# Autodesk Inventor assembly: Конвейр сборка
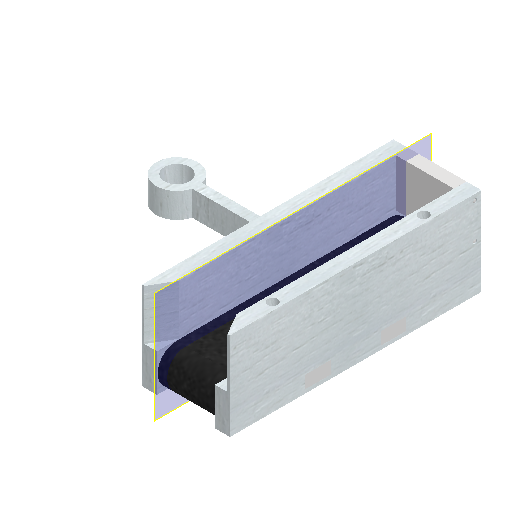
[picture p0: Inventor's stored thumbnail of the model, 512x512]
Saved by Autodesk Inventor 2022 (Build 260153000, 153)
## iProperties
Created: 2023-02-19
Part Number: Конвейр сборка
Document SubType Name: Assembly
Designer: Глеб
Mass: 469.366 g
Surface Area: 1644.22 cm^2
Volume: 465.137 cm^3
Density: 1.00909 g/cm^3
Author: Глеб
## Documents named in this file (9)
- C:\Users\Глеб\Documents\Inventor\Файлы Inventor\Конвейр сборка.iam
- C:\Users\Глеб\Documents\Inventor\Файлы Inventor\Конвейр без шпилек сборка.iam
- C:\Users\Глеб\Documents\Inventor\Файлы Inventor\Шпилька скрепления деталей.ipt
- C:\Users\Глеб\Documents\Inventor\Файлы Inventor\GearMotor\Motor.iam
- C:\Users\Глеб\Documents\Inventor\Файлы Inventor\Шкив для ДПТ.ipt
- C:\Users\Глеб\Documents\Inventor\Файлы Inventor\MX1508.ipt
- C:\Users\Глеб\Documents\Inventor\Файлы Inventor\Стенка конвейера задняя.ipt
- C:\Users\Глеб\Documents\Inventor\Файлы Inventor\Ременная передача.ipt
- C:\Users\Глеб\Documents\Inventor\Файлы Inventor\Лента конвейера.ipt
## Components (9 placed, 8 different names)
1. Лента конвейера:1 — Совмещение:25, Совмещение:26
2. Конвейр без шпилек сборка:1 [sub-assembly] — Совмещение:1, Совмещение:4, Совмещение:7, Совмещение:12, Заподлицо:8, Заподлицо:9, Заподлицо:18, Заподлицо:19, Совмещение:16, Совмещение:19, Совмещение:21, Совмещение:23, Совмещение:24, Совмещение:25
3. Шпилька скрепления деталей:1 — Совмещение:1, Заподлицо:19
4. Шпилька скрепления деталей:3 — Совмещение:4, Заподлицо:18
5. GearMotor:1 [sub-assembly] — Совмещение:16, Совмещение:18, Совмещение:19
6. Шкив для ДПТ:1 — Совмещение:15, Заподлицо:17, Совмещение:18
7. MX1508:1 — Совмещение:7, Совмещение:23, Совмещение:24
8. Стенка конвейера задняя:1 — Совмещение:12, Заподлицо:8, Заподлицо:9, Совмещение:26
9. Ременная передача:1 — Совмещение:15, Заподлицо:17, Совмещение:21
## Relationships (18: Mate 13, Flush 5)
- Совмещение:1 [Mate]: Конвейр без шпилек сборка:1 ↔ Шпилька скрепления деталей:1
- Совмещение:4 [Mate]: Конвейр без шпилек сборка:1 ↔ Шпилька скрепления деталей:3
- Совмещение:7 [Mate] (1 mm): Конвейр без шпилек сборка:1 ↔ MX1508:1
- Совмещение:12 [Mate]: Конвейр без шпилек сборка:1 ↔ Стенка конвейера задняя:1
- Заподлицо:8 [Flush]: Конвейр без шпилек сборка:1 ↔ Стенка конвейера задняя:1
- Заподлицо:9 [Flush]: Конвейр без шпилек сборка:1 ↔ Стенка конвейера задняя:1
- Совмещение:15 [Mate]: Шкив для ДПТ:1 ↔ Ременная передача:1
- Заподлицо:17 [Flush]: Шкив для ДПТ:1 ↔ Ременная передача:1
- Заподлицо:18 [Flush]: Конвейр без шпилек сборка:1 ↔ Шпилька скрепления деталей:3
- Заподлицо:19 [Flush]: Конвейр без шпилек сборка:1 ↔ Шпилька скрепления деталей:1
- Совмещение:16 [Mate] (3 mm): Конвейр без шпилек сборка:1 ↔ GearMotor:1
- Совмещение:18 [Mate]: GearMotor:1 ↔ Шкив для ДПТ:1
- Совмещение:19 [Mate] (2 mm): Конвейр без шпилек сборка:1 ↔ GearMotor:1
- Совмещение:21 [Mate]: Конвейр без шпилек сборка:1 ↔ Ременная передача:1
- Совмещение:23 [Mate] (2 mm): Конвейр без шпилек сборка:1 ↔ MX1508:1
- Совмещение:24 [Mate]: Конвейр без шпилек сборка:1 ↔ MX1508:1
- Совмещение:25 [Mate]: Лента конвейера:1 ↔ Конвейр без шпилек сборка:1
- Совмещение:26 [Mate] (0.5 mm): Лента конвейера:1 ↔ Стенка конвейера задняя:1
